# Autodesk Inventor assembly: RotaryBase
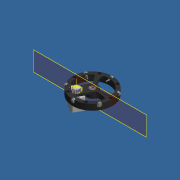
[picture p0: Inventor's stored thumbnail of the model, 180x180]
Saved by Autodesk Inventor 2014 SP2 (Build 180246200, 246)
## iProperties
Created: 2014-12-13
Part Number: RotaryBase
Document SubType Name: Assembly
Designer: 4ndreas
Author: 4ndreas
## Documents named in this file (8)
- C:\Users\4ndreas\Documents\Inventor\RobotARM v2\v3\RotaryBase.iam
- C:\Users\4ndreas\Documents\Inventor\Content Center Files\R2014\de-DE\DIN BEARING(1)\DIN 625 SKF - SKF 608.ipt
- C:\Users\4ndreas\Documents\Inventor\Content Center Files\R2014\de-DE\DIN BEARING(1)\DIN 625 SKF - SKF 625.ipt
- C:\Users\4ndreas\Documents\Inventor\Content Center Files\R2014\de-DE\DIN 931-1\DIN 931-1 - M5 x 25.ipt
- C:\Users\4ndreas\Documents\Inventor\Content Center Files\R2014\de-DE\DIN 985\DIN 985 - M5.ipt
- C:\Users\4ndreas\Documents\Inventor\RobotARM v2\Nema17.ipt
- C:\Users\4ndreas\Documents\Inventor\RobotARM v2\Stirnzahnrad_C_print.ipt
- C:\Users\4ndreas\Documents\Inventor\RobotARM v2\v3\RotaryBase_B_v2.ipt
## Components (23 placed, 7 different names)
1. RotaryBase_B_v2:1 — Fluchtend:1, Passend:1, Passend:2, Passend:3, Passend:4, Passend:5, Passend:8, Passend:9, Passend:13, Passend:16, Passend:17, Passend:18, Passend:24
2. DIN 625 SKF 608:1 — Passend:2, Passend:5
3. DIN 625 SKF 608:2 — Passend:3, Passend:4
4. Nema17:1 — Passend:16, Passend:17, Passend:18, Passend:22, Fluchtend:3
5. Stirnzahnrad_C_print:1 — Passend:22, Fluchtend:3
6. DIN 625 SKF 625:1 — Passend:8, Passend:9, Passend:10, Passend:11
7. DIN 931-1 - ersetzt durch DIN EN 24014 M5 x 25:1 — Passend:10, Passend:11, Passend:12
8. DIN 985 - ersetzt durch DIN EN ISO 10511 M5:1 — Passend:12, Passend:13
9. DIN 625 SKF 625:2
10. DIN 931-1 - ersetzt durch DIN EN 24014 M5 x 25:2
11. DIN 985 - ersetzt durch DIN EN ISO 10511 M5:2
12. DIN 625 SKF 625:3
13. DIN 931-1 - ersetzt durch DIN EN 24014 M5 x 25:3
14. DIN 985 - ersetzt durch DIN EN ISO 10511 M5:3
15. DIN 625 SKF 625:4
16. DIN 931-1 - ersetzt durch DIN EN 24014 M5 x 25:4
17. DIN 985 - ersetzt durch DIN EN ISO 10511 M5:4
18. DIN 625 SKF 625:5
19. DIN 931-1 - ersetzt durch DIN EN 24014 M5 x 25:5
20. DIN 985 - ersetzt durch DIN EN ISO 10511 M5:5
21. DIN 625 SKF 625:6
22. DIN 931-1 - ersetzt durch DIN EN 24014 M5 x 25:6
23. DIN 985 - ersetzt durch DIN EN ISO 10511 M5:6
## Component patterns: (6 elements, first: DIN 625 SKF 625:1 + DIN 931-1 - ersetzt durch DIN EN 24014 M5 x 25:1 + DIN 985 - ersetzt durch DIN EN ISO 10511 M5:1)
## Relationships (18: Mate 16, Flush 2)
- Fluchtend:1 [Flush]: RotaryBase_B_v2:1
- Passend:1 [Mate]: RotaryBase_B_v2:1
- Passend:2 [Mate]: RotaryBase_B_v2:1 ↔ DIN 625 SKF 608:1
- Passend:3 [Mate]: RotaryBase_B_v2:1 ↔ DIN 625 SKF 608:2
- Passend:4 [Mate]: RotaryBase_B_v2:1 ↔ DIN 625 SKF 608:2
- Passend:5 [Mate]: RotaryBase_B_v2:1 ↔ DIN 625 SKF 608:1
- Passend:8 [Mate]: RotaryBase_B_v2:1 ↔ DIN 625 SKF 625:1
- Passend:9 [Mate]: RotaryBase_B_v2:1 ↔ DIN 625 SKF 625:1
- Passend:10 [Mate]: DIN 625 SKF 625:1 ↔ DIN 931-1 - ersetzt durch DIN EN 24014 M5 x 25:1
- Passend:11 [Mate]: DIN 625 SKF 625:1 ↔ DIN 931-1 - ersetzt durch DIN EN 24014 M5 x 25:1
- Passend:12 [Mate]: DIN 931-1 - ersetzt durch DIN EN 24014 M5 x 25:1 ↔ DIN 985 - ersetzt durch DIN EN ISO 10511 M5:1
- Passend:13 [Mate]: RotaryBase_B_v2:1 ↔ DIN 985 - ersetzt durch DIN EN ISO 10511 M5:1
- Passend:16 [Mate]: RotaryBase_B_v2:1 ↔ Nema17:1
- Passend:17 [Mate] (9 mm): RotaryBase_B_v2:1 ↔ Nema17:1
- Passend:18 [Mate]: RotaryBase_B_v2:1 ↔ Nema17:1
- Passend:22 [Mate]: Nema17:1 ↔ Stirnzahnrad_C_print:1
- Fluchtend:3 [Flush]: Nema17:1 ↔ Stirnzahnrad_C_print:1
- Passend:24 [Mate]: RotaryBase_B_v2:1
